# Autodesk Inventor assembly: X-End-Motor v0.3
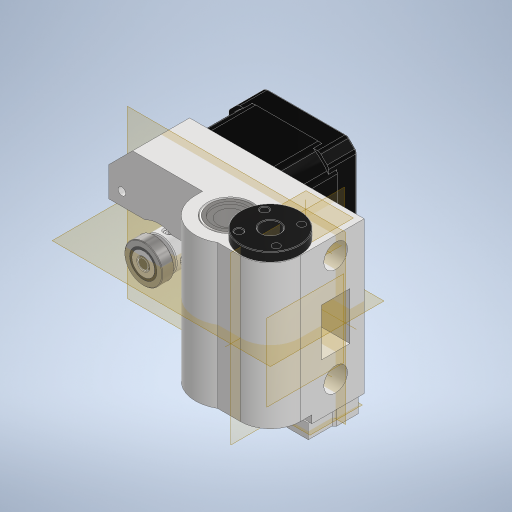
[picture p0: Inventor's stored thumbnail of the model, 512x512]
Saved by Autodesk Inventor 2023 (Build 270158000, 158)
## iProperties
Created: 2023-07-24
Part Number: X-End-Motor v0.3
Document SubType Name: Assembly
Designer: Parker
Author: Parker
## Documents named in this file (9)
- D:\000 - PEPCORP CLOUD\00- Legacy\Designs\MK3PRO P1\X-Axis\X-End-Motor v0.3.iam
- D:\000 - PEPCORP CLOUD\00- Legacy\Designs\MK3PRO P1\X-Axis\X-End-motor v0.3.ipt
- D:\000 - PEPCORP CLOUD\00- Legacy\Designs\MK3PRO P1\X-Axis\Teflon T-Nut.ipt
- D:\000 - PEPCORP CLOUD\00- Legacy\Designs\MK3PRO P1\X-Axis\x-axis-stepper-motor.iam
- D:\000 - PEPCORP CLOUD\00- Legacy\Designs\MK3PRO P1\COMPONENTS\625 Bearing.ipt
- D:\000 - PEPCORP CLOUD\00- Legacy\Designs\MK3PRO P1\COMPONENTS\LM10UU.ipt
- D:\000 - PEPCORP CLOUD\00- Legacy\Designs\MK3PRO P1\COMPONENTS\GT2_16T.ipt
- D:\000 - PEPCORP CLOUD\00- Legacy\Designs\MK3PRO P1\COMPONENTS\Small Limit Switch.iam
- D:\000 - PEPCORP CLOUD\00- Legacy\Designs\MK3PRO P1\COMPONENTS\SHCS_M2_10.ipt
## Components (10 placed, 8 different names)
1. X-End-motor v0.3:1 — Flush:1, Flush:2, Flush:3, Mate:1, Mate:2, Mate:3, Mate:4, Mate:5, Flush:5, Mate:6, Mate:8, Mate:9, Mate:12, Mate:13, Mate:14
2. Teflon T-Nut:1 — Mate:8, Mate:9
3. x-axis-stepper-motor:1 [sub-assembly] — Mate:1, Mate:2, Mate:3, Flush:4, Mate:10, Mate:11
4. 625 Bearing:1 — Mate:4, Flush:4
5. LM10UU:1 — Mate:6, Mate:7
6. LM10UU:2 — Mate:5, Flush:5, Mate:7
7. GT2_16T:1 — Mate:10, Mate:11
8. Small Limit Switch:1 [sub-assembly] — Mate:12, Mate:13, Mate:14, Mate:15, Mate:16, Mate:17, Mate:18
9. SHCS_M2_10:1 — Mate:16, Mate:17
10. SHCS_M2_10:2 — Mate:15, Mate:18
## Relationships (23: Mate 18, Flush 5)
- Flush:1: X-End-motor v0.3:1
- Flush:2: X-End-motor v0.3:1
- Flush:3: X-End-motor v0.3:1
- Mate:1: X-End-motor v0.3:1 ↔ x-axis-stepper-motor:1
- Mate:2: X-End-motor v0.3:1 ↔ x-axis-stepper-motor:1
- Mate:3: X-End-motor v0.3:1 ↔ x-axis-stepper-motor:1
- Mate:4: X-End-motor v0.3:1 ↔ 625 Bearing:1
- Flush:4: x-axis-stepper-motor:1 ↔ 625 Bearing:1
- Mate:5: X-End-motor v0.3:1 ↔ LM10UU:2
- Flush:5: X-End-motor v0.3:1 ↔ LM10UU:2
- Mate:6: X-End-motor v0.3:1 ↔ LM10UU:1
- Mate:7: LM10UU:1 ↔ LM10UU:2
- Mate:8: X-End-motor v0.3:1 ↔ Teflon T-Nut:1
- Mate:9: X-End-motor v0.3:1 ↔ Teflon T-Nut:1
- Mate:10 (0.5 mm): x-axis-stepper-motor:1 ↔ GT2_16T:1
- Mate:11: x-axis-stepper-motor:1 ↔ GT2_16T:1
- Mate:12: X-End-motor v0.3:1 ↔ Small Limit Switch:1
- Mate:13: X-End-motor v0.3:1 ↔ Small Limit Switch:1
- Mate:14: X-End-motor v0.3:1 ↔ Small Limit Switch:1
- Mate:15: Small Limit Switch:1 ↔ SHCS_M2_10:2
- Mate:16: Small Limit Switch:1 ↔ SHCS_M2_10:1
- Mate:17: Small Limit Switch:1 ↔ SHCS_M2_10:1
- Mate:18: Small Limit Switch:1 ↔ SHCS_M2_10:2
